# Autodesk Inventor assembly: projekt
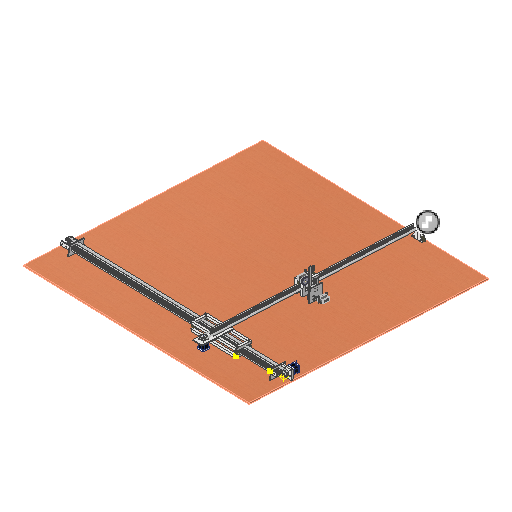
[picture p0: Inventor's stored thumbnail of the model, 512x512]
Saved by Autodesk Inventor 2025.1 (Build 291241000, 241)
## iProperties
Created: 2025-03-27
Part Number: projekt
Document SubType Name: Assembly
Designer: Maciej
Author: Maciej
## Documents named in this file (45)
- C:\Users\Maciej\Desktop\Projekt_przej-ciowy\PP\modele\projekt.iam
- C:\Users\Maciej\Desktop\Projekt_przej-ciowy\PP\modele\MASCHINENBAU_KITZ_25021000000000\25_02_1000(00-00-0)(0).ipt
- C:\Users\Maciej\Desktop\Projekt_przej-ciowy\PP\modele\podstawka pod silnik.ipt
- C:\Users\Maciej\Desktop\Projekt_przej-ciowy\PP\modele\podstawa.ipt
- C:\Users\Maciej\Desktop\Projekt_przej-ciowy\PP\modele\podstawka_prowadzaca.ipt
- C:\Users\Maciej\Desktop\Projekt_przej-ciowy\PP\modele\podstawka_prowadzaca_gora.ipt
- C:\Users\Maciej\Desktop\Projekt_przej-ciowy\PP\modele\wheel-for-v-slot-rail-system-1.snapshot.1\Wheel, V-slot Rail 625-2Z Bearing v4\Wheel, V-slot Rail 625-2Z Bearing v4\Wheel, V-slot Rail 625-2Z Bearing v4.iam
- C:\Users\Maciej\Desktop\Projekt_przej-ciowy\PP\modele\mocowanie_kolek.ipt
- C:\Users\Maciej\Desktop\Projekt_przej-ciowy\PP\modele\tuleja.ipt
- C:\Users\Maciej\Documents\Inventor\Content Center Files\R2025\pl-PL\ISO 4033(2)\ISO 4033 - M5 - ISO.ipt
- C:\Users\Maciej\Desktop\Projekt_przej-ciowy\PP\modele\MASCHINENBAU_KITZ_25011300000000\25_01_1300(00-00-0)(0).ipt
- C:\Users\Maciej\Desktop\Projekt_przej-ciowy\PP\modele\MASCHINENBAU_KITZ_25500540\25_50_0540.ipt
- C:\Users\Maciej\Documents\Inventor\Content Center Files\R2025\pl-PL\ISO 1580\ISO 1580 - M3 x 10_.ipt
- C:\Users\Maciej\Desktop\Projekt_przej-ciowy\PP\modele\stepper-motor-107.snapshot.4\Stepper Motor\Stepper Motor\Stepper Motor.ipt
- C:\Users\Maciej\Documents\Inventor\Content Center Files\R2025\pl-PL\ISO 1580\ISO 1580 - M3 x 12_.ipt
- C:\Users\Maciej\Desktop\Projekt_przej-ciowy\PP\modele\mocowanie_kolek_2.ipt
- C:\Users\Maciej\Desktop\Projekt_przej-ciowy\PP\modele\płytka_prowadzaca_rysik.ipt
- C:\Users\Maciej\Desktop\PP\modele\wheel-for-v-slot-rail-system-1.snapshot.1\Wheel, V-slot Rail 625-2Z Bearing v4\Wheel, V-slot Rail 625-2Z Bearing v4\Wheel, V-slot Rail 625-2Z Bearing v4.iam
- C:\Users\Maciej\Desktop\Projekt_przej-ciowy\PP\modele\równoważnia.ipt
- C:\Users\Maciej\Desktop\Projekt_przej-ciowy\PP\modele\tuleja_dół.ipt
- C:\Users\Maciej\Documents\Inventor\Content Center Files\R2025\pl-PL\ISO 4014(2)\ISO 4014 - M4 x 25 - ISO.ipt
- C:\Users\Maciej\Documents\Inventor\Content Center Files\R2025\pl-PL\ISO 4032(2)\ISO 4032 - M4 - ISO.ipt
- C:\Users\Maciej\Documents\Inventor\Content Center Files\R2025\pl-PL\PN-85 M-82105 B\PN-85_M-82105 - M 4 x 60 - 0,7.ipt
- C:\Users\Maciej\Desktop\Projekt_przej-ciowy\PP\modele\tuleja_gora.ipt
- C:\Users\Maciej\Desktop\PP\modele\HIWIN_20250409_215451\MGNR09R70HM_FILE_1\MGNR09R70HM_FILE_1\MGNR09R70HM_FILE_1.iam
- C:\Users\Maciej\Desktop\Projekt_przej-ciowy\PP\modele\HIWIN_20250409_220912\MGN09HZFCM_FILE_1\MGN09HZFCM_FILE_1\MGN09HZFCM_FILE_1.iam
- C:\Users\Maciej\Desktop\Projekt_przej-ciowy\PP\modele\mg-995-2.snapshot.2\Mg995\Mg995\Mg995.ipt
- C:\Users\Maciej\Desktop\Projekt_przej-ciowy\PP\modele\podstawa_rysika.ipt
- C:\Users\Maciej\Desktop\Projekt_przej-ciowy\PP\modele\lopatka.ipt
- C:\Users\Maciej\Desktop\Projekt_przej-ciowy\PP\modele\Gear.ipt
- C:\Users\Maciej\Desktop\Projekt_przej-ciowy\PP\modele\Rack.ipt
- C:\Users\Maciej\Documents\Inventor\Content Center Files\R2025\pl-PL\PN-86 M-82208  H\PN-86_M-82208 - M 2 x 8 H - 0,4.ipt
- C:\Users\Maciej\Documents\Inventor\Content Center Files\R2025\pl-PL\ISO 4762(2)\ISO 4762 - M3 x 12ISO.ipt
- C:\Users\Maciej\Documents\Inventor\Content Center Files\R2025\pl-PL\ISO 4032(2)\ISO 4032 - M3 - ISO.ipt
- C:\Users\Maciej\Desktop\Projekt_przej-ciowy\PP\modele\stol.ipt
- C:\Users\Maciej\Desktop\Projekt_przej-ciowy\PP\modele\AIS2024\42025144.iam
- C:\Users\Maciej\Desktop\Projekt_przej-ciowy\PP\modele\161727138-9-skf_bearing_k_3x5x7_tn_2\skf_bearing_k_3x5x7_tn_2.iam
- C:\Users\Maciej\Desktop\Projekt_przej-ciowy\PP\modele\tulejkapodlozysko.ipt
- C:\Users\Maciej\Desktop\Projekt_przej-ciowy\PP\modele\tulejapodlozysko_2.ipt
- C:\Users\Maciej\Desktop\Projekt_przej-ciowy\PP\modele\pasek_1.ipt
- C:\Users\Maciej\Desktop\Projekt_przej-ciowy\PP\modele\161865640-9-skf_bearing_ba_3_2\skf_bearing_ba_3_2.iam
- C:\Users\Maciej\Desktop\Projekt_przej-ciowy\PP\modele\Wał1.ipt
- C:\Users\Maciej\Documents\Inventor\Content Center Files\R2025\pl-PL\DIN 471(3)\DIN 471 - 3 x 0,4.ipt
- C:\Users\Maciej\Documents\Inventor\Content Center Files\R2025\pl-PL\DIN 471(3)\DIN 471 - 5 x 0,6.ipt
- C:\Users\Maciej\Desktop\Projekt_przej-ciowy\PP\modele\pasek_2.ipt
## Components (125 placed, 43 different names)
1. 25_02_1000(00-00-0)(0):1 — Zestawiające:1, Równoległe:1, Zestawiające:2, Zestawiające:3, Zestawiające:4, Zestawiające:5, Równoległe:2, Równoległe:4, Równoległe:5, Równoległe:6, Równoległe:7, Zestawiające:62, Zestawiające:64, Zestawiające:66, Równoległe:13, Zestawiające:68, Równoległe:25
2. podstawka pod silnik:1 — Zestawiające:1, Równoległe:1, Zestawiające:2, Zestawiające:52, Zestawiające:55, Zestawiające:61, Wstawiające:6, Wstawiające:7, Wstawiające:8, Wstawiające:9, Zestawiające:63, Wstawiające:10, Zestawiające:65, Wstawiające:11, Równoległe:23
3. podstawa:1 — Zestawiające:3, Zestawiające:4, Zestawiające:67, Zestawiające:69, Wstawiające:12, Wstawiające:13, Zestawiające:70, Równoległe:14, Zestawiające:173, Zestawiające:180, Zestawiające:182, Zestawiające:183, Zestawiające:186
4. podstawka_prowadzaca_gora:1 — Zestawiające:5, Równoległe:2, Zestawiające:6, Równoległe:3, Zestawiające:7, Zestawiające:9, Zestawiające:10, Zestawiające:11, Zestawiające:41, Zestawiające:43, Zestawiające:45, Zestawiające:47, Zestawiające:48, Zestawiające:49, Zestawiające:50, Zestawiające:51, Wstawiające:1, Zestawiające:58, Zestawiające:59, Zestawiające:60, Wstawiające:2, Wstawiające:3, Wstawiające:4, Wstawiające:5
5. podstawka_prowadzaca:1 — Zestawiające:6, Równoległe:3, Zestawiające:7, Zestawiające:8, Zestawiające:12, Równoległe:8, Zestawiające:13, Zestawiające:14, Zestawiające:15, Równoległe:9, Równoległe:10, Równoległe:11, Zestawiające:17, Zestawiające:22, Zestawiające:27, Zestawiające:33, Zestawiające:35, Zestawiające:37, Zestawiające:39
6. Wheel, V-slot Rail 625-2Z Bearing v4:1 [sub-assembly] — Zestawiające:8, Równoległe:4, Zestawiające:25, Zestawiające:29
7. Wheel, V-slot Rail 625-2Z Bearing v4:2 [sub-assembly] — Zestawiające:9, Równoległe:5, Zestawiające:31
8. Wheel, V-slot Rail 625-2Z Bearing v4:3 [sub-assembly] — Zestawiające:10, Równoległe:6, Zestawiające:18
9. Wheel, V-slot Rail 625-2Z Bearing v4:4 [sub-assembly] — Zestawiające:11, Równoległe:7, Zestawiające:20
10. mocowanie_kolek:1 — Zestawiające:12, Równoległe:8, Zestawiające:21, Zestawiające:23, Zestawiające:36, Zestawiające:42
11. mocowanie_kolek:2 — Zestawiające:13, Równoległe:11, Zestawiające:16, Zestawiające:19, Zestawiające:38, Zestawiające:46
12. mocowanie_kolek:3 — Zestawiające:15, Równoległe:10, Zestawiające:24, Zestawiające:28, Zestawiające:32, Zestawiające:44
13. mocowanie_kolek:4 — Zestawiające:14, Równoległe:9, Zestawiające:26, Zestawiające:30, Zestawiające:34, Zestawiające:40
14. tuleja:1 — Zestawiające:16, Zestawiające:17
15. tuleja:2 — Zestawiające:18, Zestawiające:19
16. tuleja:3 — Zestawiające:20, Zestawiające:21
17. tuleja:4 — Zestawiające:22, Zestawiające:23
18. tuleja:5 — Zestawiające:30, Zestawiające:31
19. tuleja:6 — Zestawiające:28, Zestawiające:29
20. tuleja:7 — Zestawiające:26, Zestawiające:27
21. tuleja:8 — Zestawiające:24, Zestawiające:25
22. ISO 4033 M5:1 — Zestawiające:32, Zestawiające:33
23. ISO 4033 M5:2 — Zestawiające:34, Zestawiające:35
24. ISO 4033 M5:3 — Zestawiające:36, Zestawiające:37
25. ISO 4033 M5:4 — Zestawiające:38, Zestawiające:39
26. ISO 4033 M5:5 — Zestawiające:40, Zestawiające:41
27. ISO 4033 M5:6 — Zestawiające:42, Zestawiające:43
28. ISO 4033 M5:7 — Zestawiające:44, Zestawiające:45
29. ISO 4033 M5:8 — Zestawiające:46, Zestawiające:47
30. 25_01_1300(00-00-0)(0):1 — Zestawiające:48, Zestawiające:49, Równoległe:12, Zestawiające:77, Zestawiające:78, Równoległe:15, Zestawiające:85, Zestawiające:86, Równoległe:18, Zestawiające:166, Równoległe:28
31. 25_50_0540:1 — Zestawiające:50, Zestawiające:51, Równoległe:12
32. ISO 1580 M3 x 10:1 — Wstawiające:1
33. Stepper Motor:1 — Zestawiające:52, Zestawiające:55, Zestawiające:61, Zestawiające:175
34. Stepper Motor:2 — Zestawiające:58, Zestawiające:59, Zestawiające:60, Zestawiające:176
35. ISO 1580 M3 x 12:1 — Wstawiające:2
36. ISO 1580 M3 x 12:2 — Wstawiające:3
37. ISO 1580 M3 x 12:3 — Wstawiające:4
38. ISO 1580 M3 x 12:4 — Wstawiające:5
39. ISO 1580 M3 x 12:5 — Wstawiające:6
40. ISO 1580 M3 x 12:6 — Wstawiające:7
41. ISO 1580 M3 x 12:7 — Wstawiające:8
42. ISO 1580 M3 x 12:8 — Wstawiające:9
43. 25_50_0540:2 — Zestawiające:62, Zestawiające:63
44. ISO 1580 M3 x 12:9 — Wstawiające:10
45. 25_50_0540:3 — Zestawiające:64, Zestawiające:65
46. ISO 1580 M3 x 12:10 — Wstawiające:11
47. 25_50_0540:4 — Zestawiające:66, Zestawiające:67, Równoległe:13
48. 25_50_0540:5 — Zestawiające:68, Zestawiające:69
49. ISO 1580 M3 x 12:11 — Wstawiające:12
50. ISO 1580 M3 x 12:12 — Wstawiające:13
51. mocowanie_kolek_2:1 — Zestawiające:70, Równoległe:14, Zestawiające:177, Zestawiające:178, Zestawiające:179, Zestawiające:181, Zestawiające:184, Zestawiające:185
52. płytka_prowadzaca_rysik:1 — Zestawiające:77, Równoległe:15, Równoległe:16, Równoległe:17, Zestawiające:79, Zestawiające:80, Wstawiające:21, Zestawiające:113, Wstawiające:22, Zestawiające:121, Zestawiające:122, Zestawiające:125
53. płytka_prowadzaca_rysik:2 — Zestawiające:78, Równoległe:16, Równoległe:17, Zestawiające:81, Zestawiające:82, Zestawiające:83, Zestawiające:84, Wstawiające:18, Wstawiające:19, Wstawiające:20, Zestawiające:120, Zestawiające:123, Zestawiające:124, Zestawiające:126, Zestawiające:127, Zestawiające:128, Zestawiające:131, Zestawiające:159, Zestawiające:161, Zestawiające:163, Zestawiające:165, Zestawiające:174, Zestawiające:201
54. Wheel, V-slot Rail 625-2Z Bearing v4:5 [sub-assembly] — Zestawiające:81, Zestawiające:84
55. Wheel, V-slot Rail 625-2Z Bearing v4:6 [sub-assembly] — Zestawiające:79, Zestawiające:82
56. Wheel, V-slot Rail 625-2Z Bearing v4:7 [sub-assembly] — Zestawiające:80, Zestawiające:83
57. równoważnia:1 — Zestawiające:85, Zestawiające:86, Równoległe:18, Zestawiające:87, Zestawiające:88, Zestawiające:89, Zestawiające:90, Zestawiające:91, Zestawiające:92, Zestawiające:93, Zestawiające:94, Wstawiające:14, Wstawiające:15, Zestawiające:100, Zestawiające:102, Zestawiające:167, Wstawiające:29, Równoległe:24, Zestawiające:200, Zestawiające:202, Zestawiające:203, Zestawiające:207
58. Wheel, V-slot Rail 625-2Z Bearing v4:8 [sub-assembly] — Zestawiające:95, Zestawiające:96
59. Wheel, V-slot Rail 625-2Z Bearing v4:9 [sub-assembly] — Zestawiające:97, Zestawiające:98
60. tuleja_dół:1 — Zestawiające:87, Zestawiające:94, Zestawiające:96
61. tuleja_dół:2 — Zestawiające:88, Zestawiające:93
62. tuleja_dół:3 — Zestawiające:89, Zestawiające:92
63. tuleja_dół:4 — Zestawiające:90, Zestawiające:91, Zestawiające:98
64. ISO 4014 M4 x 25:1 — Wstawiające:14, Zestawiające:95, Zestawiające:99
65. ISO 4014 M4 x 25:2 — Wstawiające:15, Zestawiające:97, Zestawiające:101
66. ISO 4032 M4:1 — Zestawiające:99, Zestawiające:100
67. ISO 4032 M4:2 — Zestawiające:101, Zestawiające:102
68. PN-85/M-82105 Klasa B M 4 x 60:1 — Wstawiające:18, Zestawiające:112, Zestawiające:114, Zestawiające:115
69. PN-85/M-82105 Klasa B M 4 x 60:2 — Wstawiające:19, Zestawiające:116, Zestawiające:117
70. PN-85/M-82105 Klasa B M 4 x 60:3 — Wstawiające:20, Zestawiające:118, Zestawiające:119
71. ISO 4032 M4:5 — Wstawiające:21
72. ISO 4032 M4:6 — Zestawiające:112, Zestawiające:113
73. ISO 4032 M4:7 — Wstawiające:22
74. tuleja_gora:1 — Zestawiające:118, Zestawiające:124
75. tuleja_gora:2 — Zestawiające:119, Zestawiające:125
76. tuleja_gora:3 — Zestawiające:117, Zestawiające:120
77. tuleja_gora:4 — Zestawiające:114, Zestawiające:122
78. tuleja_gora:5 — Zestawiające:115, Zestawiające:123
79. tuleja_gora:6 — Zestawiające:116, Zestawiające:121
80. MGNR09R70HM_FILE_1:1 [sub-assembly] — Zestawiające:126, Zestawiające:127, Zestawiające:128, Zestawiające:129, Zestawiające:130
81. MGN09HZFCM_FILE_1:1 [sub-assembly] — Zestawiające:129, Zestawiające:130, Zestawiające:132, Zestawiające:136, Zestawiające:137
82. Mg995:1 — Zestawiające:131, Zestawiające:140, Zestawiające:146, Zestawiające:147, Wstawiające:23, Zestawiające:148, Zestawiające:149, Wstawiające:24, Zestawiające:174, Zestawiające:201
83. podstawa_rysika:1 — Zestawiające:132, Zestawiające:133, Zestawiające:136, Zestawiające:137, Zestawiające:138, Zestawiające:139, Zestawiające:141, Równoległe:19, Równoległe:20, Zestawiające:142, Zestawiające:143, Zestawiające:144, Zestawiające:145, Zestawiające:151, Zestawiające:153, Zestawiające:155, Zestawiające:157
84. Mg995:2 — Zestawiające:133, Zestawiające:134, Zestawiające:135, Zestawiające:138, Zestawiające:139, Wstawiające:25, Wstawiające:26, Wstawiające:27, Wstawiające:28
85. lopatka:1 — Zestawiające:134, Zestawiające:135
86. Gear:1 — Zestawiające:140, Równoległe:21
87. Rack:1 — Zestawiające:141, Równoległe:19, Równoległe:20, Równoległe:21
88. PN-86/M-82208 H M 2 x 8 H:1 — Zestawiające:142
89. PN-86/M-82208 H M 2 x 8 H:2 — Zestawiające:143
90. PN-86/M-82208 H M 2 x 8 H:3 — Zestawiające:144
91. PN-86/M-82208 H M 2 x 8 H:4 — Zestawiające:145
92. ISO 4762 M3 x 12:1 — Zestawiające:146, Zestawiające:147, Zestawiające:158
93. ISO 4762 M3 x 12:2 — Wstawiające:23, Zestawiające:160
94. ISO 4762 M3 x 12:3 — Zestawiające:148, Zestawiające:149, Zestawiające:162
95. ISO 4762 M3 x 12:4 — Wstawiające:24, Zestawiające:164
96. ISO 4762 M3 x 12:5 — Wstawiające:25, Zestawiające:154
97. ISO 4762 M3 x 12:6 — Wstawiające:26, Zestawiające:156
98. ISO 4762 M3 x 12:7 — Wstawiające:27, Zestawiające:150
99. ISO 4762 M3 x 12:8 — Wstawiające:28, Zestawiające:152
100. ISO 4032 M3:1 — Zestawiające:150, Zestawiające:151
101. ISO 4032 M3:2 — Zestawiające:152, Zestawiające:153
102. ISO 4032 M3:3 — Zestawiające:154, Zestawiające:155
103. ISO 4032 M3:4 — Zestawiające:156, Zestawiające:157
104. ISO 4032 M3:5 — Zestawiające:158, Zestawiające:159
105. ISO 4032 M3:6 — Zestawiające:160, Zestawiające:161
106. ISO 4032 M3:7 — Zestawiające:162, Zestawiające:163
107. ISO 4032 M3:8 — Zestawiające:164, Zestawiające:165
108. 25_50_0540:6 — Zestawiające:166, Zestawiające:167
109. ISO 1580 M3 x 12:13 — Wstawiające:29
110. stol:1 — Zestawiające:173, Równoległe:23, Równoległe:24
111. 42025144:1 [sub-assembly] — Zestawiające:175, Równoległe:25, Równoległe:26, Zestawiające:198, Zestawiające:199
112. 42025144:2 [sub-assembly] — Zestawiające:176, Zestawiające:211
113. 42025144:3 [sub-assembly] — Zestawiające:177, Równoległe:26, Równoległe:27
114. skf_bearing_k_3x5x7_tn_2:1 [sub-assembly] — Zestawiające:178, Równoległe:27
115. ISO 4032 M3:9 — Zestawiające:179, Zestawiające:180
116. ISO 4032 M3:10 — Zestawiające:181, Zestawiające:182
117. tulejkapodlozysko:1 — Zestawiające:183, Zestawiające:184
118. tulejapodlozysko_2:1 — Zestawiające:185, Zestawiające:186
119. pasek_1:1 — Zestawiające:198, Zestawiające:199
120. 42025144:4 [sub-assembly] — Zestawiające:200, Równoległe:28, Zestawiające:210
121. skf_bearing_ba_3_2:1 [sub-assembly] — Zestawiające:202, Zestawiające:203, Zestawiające:204, Zestawiające:205
122. Wał:1 — Zestawiające:204, Zestawiające:205, Zestawiające:206, Zestawiające:208, Zestawiające:209
123. DIN 471 <= 9mm 3 x 0,4:1 — Zestawiające:206, Zestawiające:207
124. DIN 471 <= 9mm 5 x 0,6:1 — Zestawiające:208, Zestawiające:209
125. pasek_2:1 — Zestawiające:210, Zestawiające:211
## Relationships (230: Mate 176, Flush 27, Insert 27)
- Zestawiające:1 [Mate]: 25_02_1000(00-00-0)(0):1 ↔ podstawka pod silnik:1
- Równoległe:1 [Flush] (5 mm): 25_02_1000(00-00-0)(0):1 ↔ podstawka pod silnik:1
- Zestawiające:2 [Mate]: 25_02_1000(00-00-0)(0):1 ↔ podstawka pod silnik:1
- Zestawiające:3 [Mate]: 25_02_1000(00-00-0)(0):1 ↔ podstawa:1
- Zestawiające:4 [Mate]: 25_02_1000(00-00-0)(0):1 ↔ podstawa:1
- Zestawiające:5 [Mate]: 25_02_1000(00-00-0)(0):1 ↔ podstawka_prowadzaca_gora:1
- Równoległe:2 [Flush] (-25 mm): 25_02_1000(00-00-0)(0):1 ↔ podstawka_prowadzaca_gora:1
- Zestawiające:6 [Mate] (25 mm): podstawka_prowadzaca_gora:1 ↔ podstawka_prowadzaca:1
- Równoległe:3 [Flush]: podstawka_prowadzaca_gora:1 ↔ podstawka_prowadzaca:1
- Zestawiające:7 [Mate]: podstawka_prowadzaca_gora:1 ↔ podstawka_prowadzaca:1
- Zestawiające:8 [Mate]: podstawka_prowadzaca:1 ↔ Wheel, V-slot Rail 625-2Z Bearing v4:1
- Równoległe:4 [Flush] (6.95 mm): 25_02_1000(00-00-0)(0):1 ↔ Wheel, V-slot Rail 625-2Z Bearing v4:1
- Zestawiające:9 [Mate]: podstawka_prowadzaca_gora:1 ↔ Wheel, V-slot Rail 625-2Z Bearing v4:2
- Zestawiające:10 [Mate]: podstawka_prowadzaca_gora:1 ↔ Wheel, V-slot Rail 625-2Z Bearing v4:3
- Zestawiające:11 [Mate]: podstawka_prowadzaca_gora:1 ↔ Wheel, V-slot Rail 625-2Z Bearing v4:4
- Równoległe:5 [Flush] (6.95 mm): 25_02_1000(00-00-0)(0):1 ↔ Wheel, V-slot Rail 625-2Z Bearing v4:2
- Równoległe:6 [Flush] (6.95 mm): 25_02_1000(00-00-0)(0):1 ↔ Wheel, V-slot Rail 625-2Z Bearing v4:3
- Równoległe:7 [Flush] (6.95 mm): 25_02_1000(00-00-0)(0):1 ↔ Wheel, V-slot Rail 625-2Z Bearing v4:4
- Zestawiające:12 [Mate]: podstawka_prowadzaca:1 ↔ mocowanie_kolek:1
- Równoległe:8 [Flush] (-7.5 mm): podstawka_prowadzaca:1 ↔ mocowanie_kolek:1
- Zestawiające:13 [Mate]: podstawka_prowadzaca:1 ↔ mocowanie_kolek:2
- Zestawiające:14 [Mate]: podstawka_prowadzaca:1 ↔ mocowanie_kolek:4
- Zestawiające:15 [Mate]: podstawka_prowadzaca:1 ↔ mocowanie_kolek:3
- Równoległe:9 [Flush] (-7.5 mm): podstawka_prowadzaca:1 ↔ mocowanie_kolek:4
- Równoległe:10 [Flush] (-7.5 mm): podstawka_prowadzaca:1 ↔ mocowanie_kolek:3
- Równoległe:11 [Flush] (-7.5 mm): podstawka_prowadzaca:1 ↔ mocowanie_kolek:2
- Zestawiające:16 [Mate]: mocowanie_kolek:2 ↔ tuleja:1
- Zestawiające:17 [Mate]: podstawka_prowadzaca:1 ↔ tuleja:1
- Zestawiające:18 [Mate]: Wheel, V-slot Rail 625-2Z Bearing v4:3 ↔ tuleja:2
- Zestawiające:19 [Mate]: mocowanie_kolek:2 ↔ tuleja:2
- Zestawiające:20 [Mate]: Wheel, V-slot Rail 625-2Z Bearing v4:4 ↔ tuleja:3
- Zestawiające:21 [Mate]: mocowanie_kolek:1 ↔ tuleja:3
- Zestawiające:22 [Mate]: podstawka_prowadzaca:1 ↔ tuleja:4
- Zestawiające:23 [Mate]: mocowanie_kolek:1 ↔ tuleja:4
- Zestawiające:24 [Mate]: mocowanie_kolek:3 ↔ tuleja:8
- Zestawiające:25 [Mate]: Wheel, V-slot Rail 625-2Z Bearing v4:1 ↔ tuleja:8
- Zestawiające:26 [Mate]: mocowanie_kolek:4 ↔ tuleja:7
- Zestawiające:27 [Mate]: podstawka_prowadzaca:1 ↔ tuleja:7
- Zestawiające:28 [Mate]: mocowanie_kolek:3 ↔ tuleja:6
- Zestawiające:29 [Mate]: Wheel, V-slot Rail 625-2Z Bearing v4:1 ↔ tuleja:6
- Zestawiające:30 [Mate]: mocowanie_kolek:4 ↔ tuleja:5
- Zestawiające:31 [Mate]: Wheel, V-slot Rail 625-2Z Bearing v4:2 ↔ tuleja:5
- Zestawiające:32 [Mate]: mocowanie_kolek:3 ↔ ISO 4033 M5:1
- Zestawiające:33 [Mate]: podstawka_prowadzaca:1 ↔ ISO 4033 M5:1
- Zestawiające:34 [Mate]: mocowanie_kolek:4 ↔ ISO 4033 M5:2
- Zestawiające:35 [Mate]: podstawka_prowadzaca:1 ↔ ISO 4033 M5:2
- Zestawiające:36 [Mate]: mocowanie_kolek:1 ↔ ISO 4033 M5:3
- Zestawiające:37 [Mate]: podstawka_prowadzaca:1 ↔ ISO 4033 M5:3
- Zestawiające:38 [Mate]: mocowanie_kolek:2 ↔ ISO 4033 M5:4
- Zestawiające:39 [Mate]: podstawka_prowadzaca:1 ↔ ISO 4033 M5:4
- Zestawiające:40 [Mate]: mocowanie_kolek:4 ↔ ISO 4033 M5:5
- Zestawiające:41 [Mate]: podstawka_prowadzaca_gora:1 ↔ ISO 4033 M5:5
- Zestawiające:42 [Mate]: mocowanie_kolek:1 ↔ ISO 4033 M5:6
- Zestawiające:43 [Mate]: podstawka_prowadzaca_gora:1 ↔ ISO 4033 M5:6
- Zestawiające:44 [Mate]: mocowanie_kolek:3 ↔ ISO 4033 M5:7
- Zestawiające:45 [Mate]: podstawka_prowadzaca_gora:1 ↔ ISO 4033 M5:7
- Zestawiające:46 [Mate]: mocowanie_kolek:2 ↔ ISO 4033 M5:8
- Zestawiające:47 [Mate]: podstawka_prowadzaca_gora:1 ↔ ISO 4033 M5:8
- Zestawiające:48 [Mate]: podstawka_prowadzaca_gora:1 ↔ 25_01_1300(00-00-0)(0):1
- Zestawiające:49 [Mate]: podstawka_prowadzaca_gora:1 ↔ 25_01_1300(00-00-0)(0):1
- Zestawiające:50 [Mate] (2 mm): podstawka_prowadzaca_gora:1 ↔ 25_50_0540:1
- Zestawiające:51 [Mate]: podstawka_prowadzaca_gora:1 ↔ 25_50_0540:1
- Wstawiające:1 [Insert]: podstawka_prowadzaca_gora:1 ↔ ISO 1580 M3 x 10:1
- Równoległe:12 [Flush]: 25_01_1300(00-00-0)(0):1 ↔ 25_50_0540:1
- Zestawiające:52 [Mate]: podstawka pod silnik:1 ↔ Stepper Motor:1
- Zestawiające:55 [Mate]: podstawka pod silnik:1 ↔ Stepper Motor:1
- Zestawiające:58 [Mate]: podstawka_prowadzaca_gora:1 ↔ Stepper Motor:2
- Zestawiające:59 [Mate]: podstawka_prowadzaca_gora:1 ↔ Stepper Motor:2
- Zestawiające:60 [Mate]: podstawka_prowadzaca_gora:1 ↔ Stepper Motor:2
- Wstawiające:2 [Insert]: podstawka_prowadzaca_gora:1 ↔ ISO 1580 M3 x 12:1
- Wstawiające:3 [Insert]: podstawka_prowadzaca_gora:1 ↔ ISO 1580 M3 x 12:2
- Wstawiające:4 [Insert]: podstawka_prowadzaca_gora:1 ↔ ISO 1580 M3 x 12:3
- Wstawiające:5 [Insert]: podstawka_prowadzaca_gora:1 ↔ ISO 1580 M3 x 12:4
- Zestawiające:61 [Mate]: podstawka pod silnik:1 ↔ Stepper Motor:1
- Wstawiające:6 [Insert]: podstawka pod silnik:1 ↔ ISO 1580 M3 x 12:5
- Wstawiające:7 [Insert]: podstawka pod silnik:1 ↔ ISO 1580 M3 x 12:6
- Wstawiające:8 [Insert]: podstawka pod silnik:1 ↔ ISO 1580 M3 x 12:7
- Wstawiające:9 [Insert]: podstawka pod silnik:1 ↔ ISO 1580 M3 x 12:8
- Zestawiające:62 [Mate]: 25_02_1000(00-00-0)(0):1 ↔ 25_50_0540:2
- Zestawiające:63 [Mate]: podstawka pod silnik:1 ↔ 25_50_0540:2
- Wstawiające:10 [Insert]: podstawka pod silnik:1 ↔ ISO 1580 M3 x 12:9
- Zestawiające:64 [Mate]: 25_02_1000(00-00-0)(0):1 ↔ 25_50_0540:3
- Zestawiające:65 [Mate]: podstawka pod silnik:1 ↔ 25_50_0540:3
- Wstawiające:11 [Insert]: podstawka pod silnik:1 ↔ ISO 1580 M3 x 12:10
- Zestawiające:66 [Mate]: 25_02_1000(00-00-0)(0):1 ↔ 25_50_0540:4
- Zestawiające:67 [Mate]: podstawa:1 ↔ 25_50_0540:4
- Równoległe:13 [Flush]: 25_02_1000(00-00-0)(0):1 ↔ 25_50_0540:4
- Zestawiające:68 [Mate]: 25_02_1000(00-00-0)(0):1 ↔ 25_50_0540:5
- Zestawiające:69 [Mate]: podstawa:1 ↔ 25_50_0540:5
- Wstawiające:12 [Insert]: podstawa:1 ↔ ISO 1580 M3 x 12:11
- Wstawiające:13 [Insert]: podstawa:1 ↔ ISO 1580 M3 x 12:12
- Zestawiające:70 [Mate]: podstawa:1 ↔ mocowanie_kolek_2:1
- Równoległe:14 [Flush] (4 mm): podstawa:1 ↔ mocowanie_kolek_2:1
- Zestawiające:77 [Mate]: 25_01_1300(00-00-0)(0):1 ↔ płytka_prowadzaca_rysik:1
- Zestawiające:78 [Mate]: 25_01_1300(00-00-0)(0):1 ↔ płytka_prowadzaca_rysik:2
- Równoległe:15 [Flush]: 25_01_1300(00-00-0)(0):1 ↔ płytka_prowadzaca_rysik:1
- Równoległe:16 [Flush]: płytka_prowadzaca_rysik:1 ↔ płytka_prowadzaca_rysik:2
- Równoległe:17 [Flush]: płytka_prowadzaca_rysik:1 ↔ płytka_prowadzaca_rysik:2
- Zestawiające:79 [Mate]: płytka_prowadzaca_rysik:1 ↔ Wheel, V-slot Rail 625-2Z Bearing v4:6
- Zestawiające:80 [Mate]: płytka_prowadzaca_rysik:1 ↔ Wheel, V-slot Rail 625-2Z Bearing v4:7
- Zestawiające:81 [Mate]: płytka_prowadzaca_rysik:2 ↔ Wheel, V-slot Rail 625-2Z Bearing v4:5
- Zestawiające:82 [Mate] (7.4 mm): płytka_prowadzaca_rysik:2 ↔ Wheel, V-slot Rail 625-2Z Bearing v4:6
- Zestawiające:83 [Mate] (7.4 mm): płytka_prowadzaca_rysik:2 ↔ Wheel, V-slot Rail 625-2Z Bearing v4:7
- Zestawiające:84 [Mate] (7.4 mm): płytka_prowadzaca_rysik:2 ↔ Wheel, V-slot Rail 625-2Z Bearing v4:5
- Zestawiające:85 [Mate]: 25_01_1300(00-00-0)(0):1 ↔ równoważnia:1
- Zestawiające:86 [Mate]: 25_01_1300(00-00-0)(0):1 ↔ równoważnia:1
- Równoległe:18 [Flush] (1.76 mm): 25_01_1300(00-00-0)(0):1 ↔ równoważnia:1
- Zestawiające:87 [Mate]: równoważnia:1 ↔ tuleja_dół:1
- Zestawiające:88 [Mate]: równoważnia:1 ↔ tuleja_dół:2
- Zestawiające:89 [Mate]: równoważnia:1 ↔ tuleja_dół:3
- Zestawiające:90 [Mate]: równoważnia:1 ↔ tuleja_dół:4
- Zestawiające:91 [Mate]: równoważnia:1 ↔ tuleja_dół:4
- Zestawiające:92 [Mate]: równoważnia:1 ↔ tuleja_dół:3
- Zestawiające:93 [Mate]: równoważnia:1 ↔ tuleja_dół:2
- Zestawiające:94 [Mate]: równoważnia:1 ↔ tuleja_dół:1
- Wstawiające:14 [Insert]: równoważnia:1 ↔ ISO 4014 M4 x 25:1
- Wstawiające:15 [Insert]: równoważnia:1 ↔ ISO 4014 M4 x 25:2
- Zestawiające:95 [Mate]: Wheel, V-slot Rail 625-2Z Bearing v4:8 ↔ ISO 4014 M4 x 25:1
- Zestawiające:96 [Mate]: Wheel, V-slot Rail 625-2Z Bearing v4:8 ↔ tuleja_dół:1
- Zestawiające:97 [Mate]: Wheel, V-slot Rail 625-2Z Bearing v4:9 ↔ ISO 4014 M4 x 25:2
- Zestawiające:98 [Mate]: Wheel, V-slot Rail 625-2Z Bearing v4:9 ↔ tuleja_dół:4
- Zestawiające:99 [Mate]: ISO 4014 M4 x 25:1 ↔ ISO 4032 M4:1
- Zestawiające:100 [Mate]: równoważnia:1 ↔ ISO 4032 M4:1
- Zestawiające:101 [Mate]: ISO 4014 M4 x 25:2 ↔ ISO 4032 M4:2
- Zestawiające:102 [Mate]: równoważnia:1 ↔ ISO 4032 M4:2
- Wstawiające:18 [Insert]: płytka_prowadzaca_rysik:2 ↔ PN-85/M-82105 Klasa B M 4 x 60:1
- Wstawiające:19 [Insert]: płytka_prowadzaca_rysik:2 ↔ PN-85/M-82105 Klasa B M 4 x 60:2
- Wstawiające:20 [Insert]: płytka_prowadzaca_rysik:2 ↔ PN-85/M-82105 Klasa B M 4 x 60:3
- Wstawiające:21 [Insert]: płytka_prowadzaca_rysik:1 ↔ ISO 4032 M4:5
- Zestawiające:112 [Mate]: PN-85/M-82105 Klasa B M 4 x 60:1 ↔ ISO 4032 M4:6
- Zestawiające:113 [Mate]: płytka_prowadzaca_rysik:1 ↔ ISO 4032 M4:6
- Wstawiające:22 [Insert]: płytka_prowadzaca_rysik:1 ↔ ISO 4032 M4:7
- Zestawiające:114 [Mate]: PN-85/M-82105 Klasa B M 4 x 60:1 ↔ tuleja_gora:4
- Zestawiające:115 [Mate]: PN-85/M-82105 Klasa B M 4 x 60:1 ↔ tuleja_gora:5
- Zestawiające:116 [Mate]: PN-85/M-82105 Klasa B M 4 x 60:2 ↔ tuleja_gora:6
- Zestawiające:117 [Mate]: PN-85/M-82105 Klasa B M 4 x 60:2 ↔ tuleja_gora:3
- Zestawiające:118 [Mate]: PN-85/M-82105 Klasa B M 4 x 60:3 ↔ tuleja_gora:1
- Zestawiające:119 [Mate]: PN-85/M-82105 Klasa B M 4 x 60:3 ↔ tuleja_gora:2
- Zestawiające:120 [Mate]: płytka_prowadzaca_rysik:2 ↔ tuleja_gora:3
- Zestawiające:121 [Mate]: płytka_prowadzaca_rysik:1 ↔ tuleja_gora:6
- Zestawiające:122 [Mate]: płytka_prowadzaca_rysik:1 ↔ tuleja_gora:4
- Zestawiające:123 [Mate]: płytka_prowadzaca_rysik:2 ↔ tuleja_gora:5
- Zestawiające:124 [Mate]: płytka_prowadzaca_rysik:2 ↔ tuleja_gora:1
- Zestawiające:125 [Mate]: płytka_prowadzaca_rysik:1 ↔ tuleja_gora:2
- Zestawiające:126 [Mate]: płytka_prowadzaca_rysik:2 ↔ MGNR09R70HM_FILE_1:1
- Zestawiające:127 [Mate]: płytka_prowadzaca_rysik:2 ↔ MGNR09R70HM_FILE_1:1
- Zestawiające:128 [Mate]: płytka_prowadzaca_rysik:2 ↔ MGNR09R70HM_FILE_1:1
- Zestawiające:129 [Mate]: MGNR09R70HM_FILE_1:1 ↔ MGN09HZFCM_FILE_1:1
- Zestawiające:130 [Mate]: MGNR09R70HM_FILE_1:1 ↔ MGN09HZFCM_FILE_1:1
- Zestawiające:131 [Mate]: płytka_prowadzaca_rysik:2 ↔ Mg995:1
- Zestawiające:132 [Mate]: MGN09HZFCM_FILE_1:1 ↔ podstawa_rysika:1
- Zestawiające:133 [Mate]: podstawa_rysika:1 ↔ Mg995:2
- Zestawiające:134 [Mate]: Mg995:2 ↔ lopatka:1
- Zestawiające:135 [Mate] (1 mm): Mg995:2 ↔ lopatka:1
- Zestawiające:136 [Mate]: MGN09HZFCM_FILE_1:1 ↔ podstawa_rysika:1
- Zestawiające:137 [Mate]: MGN09HZFCM_FILE_1:1 ↔ podstawa_rysika:1
- Zestawiające:138 [Mate]: podstawa_rysika:1 ↔ Mg995:2
- Zestawiające:139 [Mate] (0.35 mm): podstawa_rysika:1 ↔ Mg995:2
- Zestawiające:140 [Mate]: Mg995:1 ↔ Gear:1
- Zestawiające:141 [Mate]: podstawa_rysika:1 ↔ Rack:1
- Równoległe:19 [Flush]: podstawa_rysika:1 ↔ Rack:1
- Równoległe:20 [Flush]: podstawa_rysika:1 ↔ Rack:1
- Równoległe:21 [Flush]: Gear:1 ↔ Rack:1
- Zestawiające:142 [Mate]: podstawa_rysika:1 ↔ PN-86/M-82208 H M 2 x 8 H:1
- Zestawiające:143 [Mate]: podstawa_rysika:1 ↔ PN-86/M-82208 H M 2 x 8 H:2
- Zestawiające:144 [Mate]: podstawa_rysika:1 ↔ PN-86/M-82208 H M 2 x 8 H:3
- Zestawiające:145 [Mate]: podstawa_rysika:1 ↔ PN-86/M-82208 H M 2 x 8 H:4
- Zestawiające:146 [Mate]: Mg995:1 ↔ ISO 4762 M3 x 12:1
- Zestawiające:147 [Mate]: Mg995:1 ↔ ISO 4762 M3 x 12:1
- Wstawiające:23 [Insert]: Mg995:1 ↔ ISO 4762 M3 x 12:2
- Zestawiające:148 [Mate]: Mg995:1 ↔ ISO 4762 M3 x 12:3
- Zestawiające:149 [Mate]: Mg995:1 ↔ ISO 4762 M3 x 12:3
- Wstawiające:24 [Insert]: Mg995:1 ↔ ISO 4762 M3 x 12:4
- Wstawiające:25 [Insert]: Mg995:2 ↔ ISO 4762 M3 x 12:5
- Wstawiające:26 [Insert]: Mg995:2 ↔ ISO 4762 M3 x 12:6
- Wstawiające:27 [Insert]: Mg995:2 ↔ ISO 4762 M3 x 12:7
- Wstawiające:28 [Insert]: Mg995:2 ↔ ISO 4762 M3 x 12:8
- Zestawiające:150 [Mate]: ISO 4762 M3 x 12:7 ↔ ISO 4032 M3:1
- Zestawiające:151 [Mate]: podstawa_rysika:1 ↔ ISO 4032 M3:1
- Zestawiające:152 [Mate]: ISO 4762 M3 x 12:8 ↔ ISO 4032 M3:2
- Zestawiające:153 [Mate]: podstawa_rysika:1 ↔ ISO 4032 M3:2
- Zestawiające:154 [Mate]: ISO 4762 M3 x 12:5 ↔ ISO 4032 M3:3
- Zestawiające:155 [Mate]: podstawa_rysika:1 ↔ ISO 4032 M3:3
- Zestawiające:156 [Mate]: ISO 4762 M3 x 12:6 ↔ ISO 4032 M3:4
- Zestawiające:157 [Mate]: podstawa_rysika:1 ↔ ISO 4032 M3:4
- Zestawiające:158 [Mate]: ISO 4762 M3 x 12:1 ↔ ISO 4032 M3:5
- Zestawiające:159 [Mate]: płytka_prowadzaca_rysik:2 ↔ ISO 4032 M3:5
- Zestawiające:160 [Mate]: ISO 4762 M3 x 12:2 ↔ ISO 4032 M3:6
- Zestawiające:161 [Mate]: płytka_prowadzaca_rysik:2 ↔ ISO 4032 M3:6
- Zestawiające:162 [Mate]: ISO 4762 M3 x 12:3 ↔ ISO 4032 M3:7
- Zestawiające:163 [Mate]: płytka_prowadzaca_rysik:2 ↔ ISO 4032 M3:7
- Zestawiające:164 [Mate]: ISO 4762 M3 x 12:4 ↔ ISO 4032 M3:8
- Zestawiające:165 [Mate]: płytka_prowadzaca_rysik:2 ↔ ISO 4032 M3:8
- Zestawiające:166 [Mate]: 25_01_1300(00-00-0)(0):1 ↔ 25_50_0540:6
- Zestawiające:167 [Mate]: równoważnia:1 ↔ 25_50_0540:6
- Wstawiające:29 [Insert]: równoważnia:1 ↔ ISO 1580 M3 x 12:13
- Zestawiające:173 [Mate]: podstawa:1 ↔ stol:1
- Równoległe:23 [Flush]: podstawka pod silnik:1 ↔ stol:1
- Równoległe:24 [Flush] (-10 mm): równoważnia:1 ↔ stol:1
- Zestawiające:174 [Mate]: płytka_prowadzaca_rysik:2 ↔ Mg995:1
- Zestawiające:175 [Mate]: Stepper Motor:1 ↔ 42025144:1
- Równoległe:25 [Flush]: 25_02_1000(00-00-0)(0):1 ↔ 42025144:1
- Zestawiające:176 [Mate]: Stepper Motor:2 ↔ 42025144:2
- Zestawiające:177 [Mate]: mocowanie_kolek_2:1 ↔ 42025144:3
- Równoległe:26 [Flush]: 42025144:1 ↔ 42025144:3
- Zestawiające:178 [Mate]: mocowanie_kolek_2:1 ↔ skf_bearing_k_3x5x7_tn_2:1
- Równoległe:27 [Flush] (5.5 mm): 42025144:3 ↔ skf_bearing_k_3x5x7_tn_2:1
- Zestawiające:179 [Mate]: mocowanie_kolek_2:1 ↔ ISO 4032 M3:9
- Zestawiające:180 [Mate]: podstawa:1 ↔ ISO 4032 M3:9
- Zestawiające:181 [Mate]: mocowanie_kolek_2:1 ↔ ISO 4032 M3:10
- Zestawiające:182 [Mate]: podstawa:1 ↔ ISO 4032 M3:10
- Zestawiające:183 [Mate]: podstawa:1 ↔ tulejkapodlozysko:1
- Zestawiające:184 [Mate]: mocowanie_kolek_2:1 ↔ tulejkapodlozysko:1
- Zestawiające:185 [Mate]: mocowanie_kolek_2:1 ↔ tulejapodlozysko_2:1
- Zestawiające:186 [Mate]: podstawa:1 ↔ tulejapodlozysko_2:1
- Zestawiające:198 [Mate]: 42025144:1 ↔ pasek_1:1
- Zestawiające:199 [Mate] (1.5 mm): 42025144:1 ↔ pasek_1:1
- Zestawiające:200 [Mate]: równoważnia:1 ↔ 42025144:4
- Równoległe:28 [Flush] (1 mm): 25_01_1300(00-00-0)(0):1 ↔ 42025144:4
- Zestawiające:201 [Mate]: płytka_prowadzaca_rysik:2 ↔ Mg995:1
- Zestawiające:202 [Mate]: równoważnia:1 ↔ skf_bearing_ba_3_2:1
- Zestawiające:203 [Mate]: równoważnia:1 ↔ skf_bearing_ba_3_2:1
- Zestawiające:204 [Mate]: skf_bearing_ba_3_2:1 ↔ Wał:1
- Zestawiające:205 [Mate]: skf_bearing_ba_3_2:1 ↔ Wał:1
- Zestawiające:206 [Mate]: Wał:1 ↔ DIN 471 <= 9mm 3 x 0,4:1
- Zestawiające:207 [Mate]: równoważnia:1 ↔ DIN 471 <= 9mm 3 x 0,4:1
- Zestawiające:208 [Mate]: Wał:1 ↔ DIN 471 <= 9mm 5 x 0,6:1
- Zestawiające:209 [Mate]: Wał:1 ↔ DIN 471 <= 9mm 5 x 0,6:1
- Zestawiające:210 [Mate]: 42025144:4 ↔ pasek_2:1
- Zestawiające:211 [Mate] (1.5 mm): 42025144:2 ↔ pasek_2:1
